# Autodesk Inventor assembly: LegRod
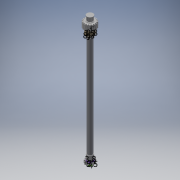
[picture p0: Inventor's stored thumbnail of the model, 180x180]
Saved by Autodesk Inventor 2019.1 (Build 231200000, 200)
## iProperties
Created: 2018-11-25
Part Number: LegRod
Material: Generisch
Document SubType Name: Assembly
Designer: JochenAlt
Author: JochenAlt
## Documents named in this file (4)
- D:\Projects\Ondine\CAD\Leg\LegRod.iam
- D:\Projects\Ondine\CAD\Leg\Stirnzahnrad21.ipt
- D:\Projects\Ondine\CAD\Spindle\SpindleWithGear.ipt
- D:\Projects\Ondine\CAD\Leg\Rod.ipt
## Components (3 placed, 3 different names)
1. Stirnzahnrad2:1 — Passend:1, Passend:2
2. Spindle:1 — Passend:3, Passend:4
3. Rod:1 — Passend:1, Passend:2, Passend:3, Passend:4
## Relationships (4: Mate 4)
- Passend:1 [Mate]: Stirnzahnrad2:1 ↔ Rod:1
- Passend:2 [Mate]: Stirnzahnrad2:1 ↔ Rod:1
- Passend:3 [Mate]: Spindle:1 ↔ Rod:1
- Passend:4 [Mate]: Spindle:1 ↔ Rod:1
